# Autodesk Inventor assembly: Assembly1
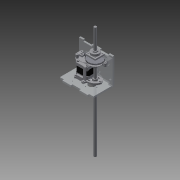
[picture p0: Inventor's stored thumbnail of the model, 180x180]
Saved by Autodesk Inventor 2015 (Build 190159000, 159)
## iProperties
Created: 2017-03-07
Part Number: Assembly1
Document SubType Name: Assembly
Designer: Ernest
Author: Ernest
## Documents named in this file (22)
- C:\Users\1esh9\Documents\Capstone-Project\doc\CAD\EndEffectorBase2\Assembly1.iam
- C:\Users\1esh9\Documents\Capstone-Project\doc\CAD\EndEffectorBase2\ThreadBar90.ipt
- C:\Users\1esh9\Documents\Capstone-Project\doc\CAD\Stepper Motor\NEMA-17\NEMA 17.iam
- C:\Users\1esh9\Documents\Capstone-Project\doc\CAD\Gears\Spur Gears1.iam
- C:\Users\1esh9\Documents\Capstone-Project\doc\CAD\Sensors\LinesensorHolderBottom.ipt
- C:\Users\1esh9\Documents\Capstone-Project\doc\CAD\Sensors\LinesensorHolderTop.ipt
- C:\Users\1esh9\Documents\Capstone-Project\doc\CAD\Sensors\LinesensorHolderWasher.ipt
- C:\Users\1esh9\Documents\Capstone-Project\doc\CAD\EndEffectorBase2\BigPositionDisk.ipt
- C:\Users\1esh9\Documents\Capstone-Project\doc\CAD\EndEffectorBase2\SmallPositionDisk.ipt
- C:\Users\1esh9\Documents\Capstone-Project\doc\CAD\LowLevel_Rev3\EE_base\EE_base_assembly.iam
- C:\Users\1esh9\Documents\Capstone-Project\doc\CAD\EndEffectorBase2\BallBearing.ipt
- C:\Users\1esh9\Documents\Capstone-Project\doc\CAD\EndEffectorBase2\BallBearingCenterer.ipt
- C:\Users\1esh9\Documents\Capstone-Project\doc\CAD\EndEffectorBase2\9mmRodNut.ipt
- C:\Users\1esh9\Documents\Capstone-Project\doc\CAD\EndEffectorBase2\BallBearingHolderTop.ipt
- C:\Users\1esh9\Documents\Capstone-Project\doc\CAD\EndEffectorBase2\BallBearingHolderBottom.ipt
- C:\Users\1esh9\Documents\Capstone-Project\doc\CAD\Sensors\TestMount.ipt
- C:\Users\1esh9\Documents\Capstone-Project\doc\CAD\EndEffectorBase2\MotorBracket.ipt
- C:\Users\1esh9\Documents\Capstone-Project\doc\CAD\Nuts and Bolts\SensorBolt-M3x11.ipt
- C:\Users\1esh9\Documents\Capstone-Project\doc\CAD\Sensors\LinesensorHolderBottomRound.ipt
- C:\Users\1esh9\Documents\Capstone-Project\doc\CAD\Sensors\LinesensorHolderTopRound.ipt
- C:\Users\1esh9\Documents\Capstone-Project\doc\CAD\Sensors\LinesensorHolderWasherRound.ipt
- C:\Users\1esh9\Documents\Capstone-Project\doc\CAD\Sensors\LinesensorHolderMidRound.ipt
## Components (33 placed, 21 different names)
1. ThreadBar90:1 — Mate:14, Mate:22, Mate:23, Mate:24, Mate:25, Mate:31, Mate:41, Mate:42, Mate:59, Mate:60, Mate:72
2. NEMA 17:1 [sub-assembly] — Mate:1, Mate:26, Mate:32, Mate:43, Mate:44, Mate:45, Mate:46, Angle:4, Mate:47, Mate:48, Mate:49, Mate:50, Mate:51, Mate:52, Mate:58
3. Spur Gears:1 [sub-assembly] — Mate:1, Mate:14, Mate:16, Mate:17, Mate:28, Mate:56
4. LinesensorHolderBottom:2 — Mate:5, Mate:6, Mate:7, Mate:43, Angle:4
5. LinesensorHolderTop:2 — Mate:2, Mate:3, Mate:4, Mate:5, Mate:7, Mate:38, Mate:39, Mate:40
6. LinesensorHolderWasher:1 — Mate:2, Mate:3, Mate:4, Mate:6
7. LinesensorHolderWasher:2 — Flush:5, Mate:59, Mate:60, Flush:7, Mate:64, Flush:8
8. BigPositionDisk:1 — Mate:31, Flush:5
9. SmallPositionDisk:1 — Mate:32, Mate:38, Mate:39, Mate:40
10. EE_base_assembly:1 [sub-assembly] — Flush:1, Mate:33, Mate:57
11. BallBearing:1 — Mate:16, Mate:20, Flush:3, Mate:27
12. BallBearing:2 — Mate:17, Flush:1, Mate:21, Flush:2, Mate:26
13. BallBearingCenterer:1 — Mate:20, Flush:3
14. BallBearingCenterer:2 — Mate:21, Flush:2
15. 9mmRodNut:1 — Mate:24
16. 9mmRodNut:2 — Mate:25
17. 9mmRodNut:3 — Mate:22
18. 9mmRodNut:4 — Mate:23
19. BallBearingHolderTop:1 — Mate:27, Mate:28, Mate:33
20. BallBearingHolderBottom:1 — Mate:56, Mate:57, Mate:58
21. 9mmRodNut:5 — Mate:41
22. 9mmRodNut:6 — Mate:42
23. TestMount:1 — Mate:44, Mate:45, Mate:46
24. MotorBracket:1 — Mate:48, Mate:50, Mate:52, Mate:55, Mate:62
25. MotorBracket:2 — Mate:47, Mate:49, Mate:51, Mate:53, Mate:54, Mate:61, Mate:63
26. SensorBolt-M3x11:1 — Flush:4, Mate:55
27. SensorBolt-M3x11:2 — Flush:4, Mate:53, Mate:54
28. SensorBolt-M3x11:3 — Flush:6, Mate:62
29. SensorBolt-M3x11:4 — Flush:6, Mate:61, Mate:63
30. LinesensorHolderBottomRound:1 — Mate:65, Mate:67, Flush:9, Mate:69, Flush:11, Mate:71
31. LinesensorHolderTopRound:1 — Mate:66, Mate:68, Flush:10, Mate:69
32. LinesensorHolderWasherRound:1 — Flush:7, Mate:64, Flush:8, Mate:65, Mate:66, Mate:67, Mate:68, Flush:9, Flush:10, Flush:11
33. LinesensorHolderMidRound:1 — Mate:71, Mate:72
## Relationships (68: Mate 56, Flush 11, Angle 1)
- Mate:1: NEMA 17:1 ↔ Spur Gears:1
- Mate:2: LinesensorHolderTop:2 ↔ LinesensorHolderWasher:1
- Mate:3: LinesensorHolderTop:2 ↔ LinesensorHolderWasher:1
- Mate:4: LinesensorHolderTop:2 ↔ LinesensorHolderWasher:1
- Mate:5: LinesensorHolderBottom:2 ↔ LinesensorHolderTop:2
- Mate:6: LinesensorHolderBottom:2 ↔ LinesensorHolderWasher:1
- Mate:7: LinesensorHolderBottom:2 ↔ LinesensorHolderTop:2
- Mate:14: ThreadBar90:1 ↔ Spur Gears:1
- Mate:16: Spur Gears:1 ↔ BallBearing:1
- Mate:17: Spur Gears:1 ↔ BallBearing:2
- Flush:1: EE_base_assembly:1 ↔ BallBearing:2
- Mate:20: BallBearing:1 ↔ BallBearingCenterer:1
- Mate:21: BallBearing:2 ↔ BallBearingCenterer:2
- Flush:2 (0.4 mm): BallBearing:2 ↔ BallBearingCenterer:2
- Flush:3 (0.4 mm): BallBearing:1 ↔ BallBearingCenterer:1
- Mate:22: ThreadBar90:1 ↔ 9mmRodNut:3
- Mate:23: ThreadBar90:1 ↔ 9mmRodNut:4
- Mate:24: ThreadBar90:1 ↔ 9mmRodNut:1
- Mate:25: ThreadBar90:1 ↔ 9mmRodNut:2
- Mate:26 (5 mm): NEMA 17:1 ↔ BallBearing:2
- Mate:27: BallBearing:1 ↔ BallBearingHolderTop:1
- Mate:28: Spur Gears:1 ↔ BallBearingHolderTop:1
- Mate:31: ThreadBar90:1 ↔ BigPositionDisk:1
- Mate:32: NEMA 17:1 ↔ SmallPositionDisk:1
- Mate:33: EE_base_assembly:1 ↔ BallBearingHolderTop:1
- Mate:38 (0.2 mm): LinesensorHolderTop:2 ↔ SmallPositionDisk:1
- Mate:39 (26.387 mm): LinesensorHolderTop:2 ↔ SmallPositionDisk:1
- Mate:40 (26.387 mm): LinesensorHolderTop:2 ↔ SmallPositionDisk:1
- Mate:41: ThreadBar90:1 ↔ 9mmRodNut:5
- Mate:42: ThreadBar90:1 ↔ 9mmRodNut:6
- Mate:43 (3 mm): NEMA 17:1 ↔ LinesensorHolderBottom:2
- Mate:44: NEMA 17:1 ↔ TestMount:1
- Mate:45: NEMA 17:1 ↔ TestMount:1
- Mate:46: NEMA 17:1 ↔ TestMount:1
- Angle:4 (0 deg): NEMA 17:1 ↔ LinesensorHolderBottom:2
- Mate:47: NEMA 17:1 ↔ MotorBracket:2
- Mate:48: NEMA 17:1 ↔ MotorBracket:1
- Mate:49: NEMA 17:1 ↔ MotorBracket:2
- Mate:50: NEMA 17:1 ↔ MotorBracket:1
- Mate:51: NEMA 17:1 ↔ MotorBracket:2
- Mate:52: NEMA 17:1 ↔ MotorBracket:1
- Flush:4: SensorBolt-M3x11:1 ↔ SensorBolt-M3x11:2
- Mate:53: MotorBracket:2 ↔ SensorBolt-M3x11:2
- Mate:54: MotorBracket:2 ↔ SensorBolt-M3x11:2
- Mate:55: MotorBracket:1 ↔ SensorBolt-M3x11:1
- Mate:56: Spur Gears:1 ↔ BallBearingHolderBottom:1
- Mate:57: EE_base_assembly:1 ↔ BallBearingHolderBottom:1
- Mate:58: NEMA 17:1 ↔ BallBearingHolderBottom:1
- Flush:5 (-0.2 mm): LinesensorHolderWasher:2 ↔ BigPositionDisk:1
- Mate:59 (26.387 mm): ThreadBar90:1 ↔ LinesensorHolderWasher:2
- Mate:60 (26.387 mm): ThreadBar90:1 ↔ LinesensorHolderWasher:2
- Flush:6: SensorBolt-M3x11:3 ↔ SensorBolt-M3x11:4
- Mate:61: MotorBracket:2 ↔ SensorBolt-M3x11:4
- Mate:62: MotorBracket:1 ↔ SensorBolt-M3x11:3
- Mate:63: MotorBracket:2 ↔ SensorBolt-M3x11:4
- Flush:7: LinesensorHolderWasher:2 ↔ LinesensorHolderWasherRound:1
- Mate:64 (3.2 mm): LinesensorHolderWasher:2 ↔ LinesensorHolderWasherRound:1
- Flush:8: LinesensorHolderWasher:2 ↔ LinesensorHolderWasherRound:1
- Mate:65: LinesensorHolderBottomRound:1 ↔ LinesensorHolderWasherRound:1
- Mate:66: LinesensorHolderTopRound:1 ↔ LinesensorHolderWasherRound:1
- Mate:67: LinesensorHolderBottomRound:1 ↔ LinesensorHolderWasherRound:1
- Mate:68: LinesensorHolderTopRound:1 ↔ LinesensorHolderWasherRound:1
- Flush:9: LinesensorHolderBottomRound:1 ↔ LinesensorHolderWasherRound:1
- Flush:10: LinesensorHolderTopRound:1 ↔ LinesensorHolderWasherRound:1
- Mate:69: LinesensorHolderBottomRound:1 ↔ LinesensorHolderTopRound:1
- Flush:11: LinesensorHolderBottomRound:1 ↔ LinesensorHolderWasherRound:1
- Mate:71: LinesensorHolderBottomRound:1 ↔ LinesensorHolderMidRound:1
- Mate:72: ThreadBar90:1 ↔ LinesensorHolderMidRound:1
